# Autodesk Inventor assembly: Robot
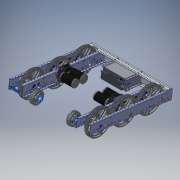
[picture p0: Inventor's stored thumbnail of the model, 180x180]
Saved by Autodesk Inventor 2016 (Build 200138000, 138)
## iProperties
Created: 2016-01-27
Part Number: Robot
Document SubType Name: Assembly
Designer: PrashantBIA
Author: PrashantBIA
## Documents named in this file (10)
- C:\Users\17swamipr\Desktop\Robot Assembly 1-27-15 v3.0 Swami\Robot Assembly\Robot.iam
- C:\Users\17swamipr\Desktop\Robot Assembly 1-27-15 v3.0 Swami\Robot Assembly\Drive Train\AM14U3+Square+REV1-1.iam
- C:\Users\17swamipr\Desktop\Robot Assembly 1-27-15 v3.0 Swami\Robot Assembly\Electronic Parts\CIM Motor.ipt
- C:\Users\17swamipr\Desktop\Robot Assembly 1-27-15 v3.0 Swami\Robot Assembly\1x1\22in.ipt
- C:\Users\17swamipr\Desktop\Robot Assembly 1-27-15 v3.0 Swami\Robot Assembly\Electronic Parts\Electrical Board Assembly.iam
- C:\Users\17swamipr\Desktop\Robot Assembly 1-27-15 v3.0 Swami\Robot Assembly\Electronic Parts\am-2939+BatteryHolder.ipt
- C:\Users\17swamipr\Desktop\Robot Assembly 1-27-15 v3.0 Swami\Robot Assembly\Electronic Parts\ELEC_Battery_NP18-12B.ipt
- C:\Users\17swamipr\Desktop\Robot Assembly 1-27-15 v3.0 Swami\Robot Assembly\Special Assemblies\8inWheel.iam
- C:\Users\17swamipr\Desktop\Robot Assembly 1-27-15 v3.0 Swami\Robot Assembly\Special Assemblies\Middle8inWheel.iam
- C:\Users\17swamipr\Desktop\Robot Assembly 1-27-15 v3.0 Swami\Robot Assembly\Special Assemblies\XWheel.iam
## Components (18 placed, 9 different names)
1. XWheel:1 [sub-assembly] — Flush:5, Mate:43, Mate:44
2. XWheel:2 [sub-assembly] — Flush:6, Mate:43, Mate:45
3. CIM Motor:4 — Insert:2
4. CIM Motor:3 — Insert:1
5. CIM Motor:2 — Insert:3
6. CIM Motor:1 — Insert:4
7. AM14U3+Square+REV1-1:1 [sub-assembly] — Insert:1, Insert:2, Flush:1, Mate:15, Mate:16, Flush:2, Mate:19, Mate:20, Mate:21, Mate:24, Mate:25, Mate:26, Mate:27, Mate:28, Mate:30, Mate:31, Mate:32, Mate:33, Mate:35, Mate:36, Mate:38, Insert:3, Insert:4, Mate:40, Mate:41, Mate:42, Flush:5, Flush:6, Mate:44, Mate:45
8. 22in:1 — Flush:1, Mate:15, Mate:17, Flush:4
9. 22in:2 — Mate:16, Flush:2, Mate:17, Flush:3, Mate:18
10. Electrical Board Assembly:1 [sub-assembly] — Flush:3, Mate:18, Flush:4
11. am-2939+BatteryHolder:1 — Mate:19, Mate:20, Mate:21, Mate:22, Mate:23
12. ELEC_Battery_NP18-12B:1 — Mate:22, Mate:23, Mate:24
13. Middle8inWheel:2 [sub-assembly] — Mate:36, Mate:42
14. Middle8inWheel:1 [sub-assembly] — Mate:35, Mate:38
15. 8inWheel:4 [sub-assembly] — Mate:28, Mate:41
16. 8inWheel:3 [sub-assembly] — Mate:32, Mate:33, Mate:40
17. 8inWheel:2 [sub-assembly] — Mate:30, Mate:31
18. 8inWheel:1 [sub-assembly] — Mate:25, Mate:26, Mate:27
## Relationships (37: Mate 27, Flush 6, Insert 4)
- Insert:1: CIM Motor:3 ↔ AM14U3+Square+REV1-1:1
- Insert:2: CIM Motor:4 ↔ AM14U3+Square+REV1-1:1
- Flush:1: AM14U3+Square+REV1-1:1 ↔ 22in:1
- Mate:15: AM14U3+Square+REV1-1:1 ↔ 22in:1
- Mate:16: AM14U3+Square+REV1-1:1 ↔ 22in:2
- Flush:2: AM14U3+Square+REV1-1:1 ↔ 22in:2
- Mate:17 (304.8 mm): 22in:1 ↔ 22in:2
- Flush:3: 22in:2 ↔ Electrical Board Assembly:1
- Mate:18: 22in:2 ↔ Electrical Board Assembly:1
- Flush:4 (-76.2 mm): 22in:1 ↔ Electrical Board Assembly:1
- Mate:19: AM14U3+Square+REV1-1:1 ↔ am-2939+BatteryHolder:1
- Mate:20: AM14U3+Square+REV1-1:1 ↔ am-2939+BatteryHolder:1
- Mate:21: AM14U3+Square+REV1-1:1 ↔ am-2939+BatteryHolder:1
- Mate:22: am-2939+BatteryHolder:1 ↔ ELEC_Battery_NP18-12B:1
- Mate:23: am-2939+BatteryHolder:1 ↔ ELEC_Battery_NP18-12B:1
- Mate:24: AM14U3+Square+REV1-1:1 ↔ ELEC_Battery_NP18-12B:1
- Mate:25: AM14U3+Square+REV1-1:1 ↔ 8inWheel:1
- Mate:26: AM14U3+Square+REV1-1:1 ↔ 8inWheel:1
- Mate:27: AM14U3+Square+REV1-1:1 ↔ 8inWheel:1
- Mate:28: AM14U3+Square+REV1-1:1 ↔ 8inWheel:4
- Mate:30: AM14U3+Square+REV1-1:1 ↔ 8inWheel:2
- Mate:31: AM14U3+Square+REV1-1:1 ↔ 8inWheel:2
- Mate:32: AM14U3+Square+REV1-1:1 ↔ 8inWheel:3
- Mate:33: AM14U3+Square+REV1-1:1 ↔ 8inWheel:3
- Mate:35: AM14U3+Square+REV1-1:1 ↔ Middle8inWheel:1
- Mate:36: AM14U3+Square+REV1-1:1 ↔ Middle8inWheel:2
- Mate:38: AM14U3+Square+REV1-1:1 ↔ Middle8inWheel:1
- Insert:3: CIM Motor:2 ↔ AM14U3+Square+REV1-1:1
- Insert:4: CIM Motor:1 ↔ AM14U3+Square+REV1-1:1
- Mate:40: AM14U3+Square+REV1-1:1 ↔ 8inWheel:3
- Mate:41: AM14U3+Square+REV1-1:1 ↔ 8inWheel:4
- Mate:42: AM14U3+Square+REV1-1:1 ↔ Middle8inWheel:2
- Flush:5: XWheel:1 ↔ AM14U3+Square+REV1-1:1
- Flush:6: XWheel:2 ↔ AM14U3+Square+REV1-1:1
- Mate:43: XWheel:1 ↔ XWheel:2
- Mate:44 (50.8 mm): XWheel:1 ↔ AM14U3+Square+REV1-1:1
- Mate:45 (50.8 mm): XWheel:2 ↔ AM14U3+Square+REV1-1:1
